# Autodesk Inventor assembly: Frame
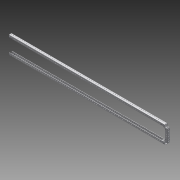
[picture p0: Inventor's stored thumbnail of the model, 180x180]
Saved by Autodesk Inventor 2014 (Build 180170000, 170)
## iProperties
Created: 2015-01-20
Part Number: Frame
Document SubType Name: Assembly
Designer: chappelled
Author: chappelled
## Documents named in this file (9)
- C:\Users\chappelled\Documents\Inventor\Claw\Frame.iam
- C:\Users\chappelled\Documents\Inventor\Claw\End Bracket.iam
- C:\Users\chappelled\Documents\Inventor\Claw\DBK_C-Channel_72.ipt
- C:\Users\chappelled\Documents\Inventor\Claw\Frame\Design Accelerator\Bolted Connection1.iam
- C:\Users\chappelled\Documents\Inventor\Claw\Frame\Design Accelerator\Bolted Connection2.iam
- C:\Users\chappelled\Documents\Inventor\Claw\Frame\Design Accelerator\Bolted Connection3.iam
- C:\Users\chappelled\Documents\Inventor\Claw\Frame\Design Accelerator\Bolted Connection4.iam
- C:\Users\chappelled\Documents\Inventor\Claw\Frame\Design Accelerator\Bolted Connection5.iam
- C:\Users\chappelled\Documents\Inventor\Claw\Frame\Design Accelerator\Bolted Connection6.iam
## Components (11 placed, 3 different names)
1. DBK_C-Channel_72:1 — Mate:4, Mate:5, Mate:6, Mate:7, Mate:22, Mate:23, Mate:24, Mate:25, Mate:26
2. Bolted Connection:1 [sub-assembly] — Mate:4, Mate:5
3. Bolted Connection:2 [sub-assembly] — Mate:6, Mate:7
4. End Bracket:2 [sub-assembly]
5. DBK_C-Channel_72:2 — Mate:18, Mate:19, Mate:20, Mate:21
6. Bolted Connection:3 [sub-assembly]
7. Bolted Connection:4 [sub-assembly]
8. Bolted Connection:5 [sub-assembly] — Mate:18, Mate:19
9. Bolted Connection:6 [sub-assembly] — Mate:20, Mate:21
10. Bolted Connection:7 [sub-assembly] — Mate:22, Mate:23
11. Bolted Connection:8 [sub-assembly] — Mate:24, Mate:25
## Relationships (20: Mate 20)
- Mate:4: DBK_C-Channel_72:1 ↔ Bolted Connection:1
- Mate:5: DBK_C-Channel_72:1 ↔ Bolted Connection:1
- Mate:6: DBK_C-Channel_72:1 ↔ Bolted Connection:2
- Mate:7: DBK_C-Channel_72:1 ↔ Bolted Connection:2
- [Mate]: End Bracket:2 ↔ DBK_C-Channel_72:2
- [Mate]: End Bracket:2 ↔ DBK_C-Channel_72:2
- [Mate]: End Bracket:2 ↔ DBK_C-Channel_72:2
- [Mate]: DBK_C-Channel_72:2 ↔ Bolted Connection:3
- [Mate]: DBK_C-Channel_72:2 ↔ Bolted Connection:3
- [Mate]: DBK_C-Channel_72:2 ↔ Bolted Connection:4
- [Mate]: DBK_C-Channel_72:2 ↔ Bolted Connection:4
- Mate:18: DBK_C-Channel_72:2 ↔ Bolted Connection:5
- Mate:19: DBK_C-Channel_72:2 ↔ Bolted Connection:5
- Mate:20: DBK_C-Channel_72:2 ↔ Bolted Connection:6
- Mate:21: DBK_C-Channel_72:2 ↔ Bolted Connection:6
- Mate:22: DBK_C-Channel_72:1 ↔ Bolted Connection:7
- Mate:23: DBK_C-Channel_72:1 ↔ Bolted Connection:7
- Mate:24: DBK_C-Channel_72:1 ↔ Bolted Connection:8
- Mate:25: DBK_C-Channel_72:1 ↔ Bolted Connection:8
- Mate:26: DBK_C-Channel_72:1
## Named parameters: d7_d5 = 0 mm, d8_d6 = 0 mm, d9_d3 = 0 mm, d10_d4 = 0 mm, d11_d2 = 0 mm, d12_d0 = 0 mm, d13_d1 = 0 mm
